# Autodesk Inventor assembly: CameraCaseMountV02
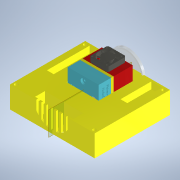
[picture p0: Inventor's stored thumbnail of the model, 180x180]
Saved by Autodesk Inventor 2022.2 (Build 262287000, 287)
## iProperties
Created: 2021-11-28
Part Number: CameraCaseMountV02
Document SubType Name: Assembly
Designer: robst
Author: robst
## Documents named in this file (4)
- C:\git\CAD-Development\robSteele\ShapeWays\GlobalMeteorNetwork\CameraCaseMountV02.iam
- C:\git\CAD-Development\robSteele\ShapeWays\GlobalMeteorNetwork\caseLowerPortionV02.ipt
- C:\git\CAD-Development\robSteele\ShapeWays\GlobalMeteorNetwork\IMX291 Camera Case Assembly.iam
- C:\git\CAD-Development\robSteele\ShapeWays\GlobalMeteorNetwork\50mmFilter.ipt
## Components (3 placed, 3 different names)
1. caseLowerPortionV02:1 — Mate:1, Mate:2, Mate:3, Insert:1
2. IMX291 Camera Case Assembly:1 [sub-assembly] — Mate:1, Mate:2, Mate:3
3. 50mmFilter:1 — Insert:1
## Relationships (4: Mate 3, Insert 1)
- Mate:1 (1 mm): caseLowerPortionV02:1 ↔ IMX291 Camera Case Assembly:1
- Mate:2 (1 mm): caseLowerPortionV02:1 ↔ IMX291 Camera Case Assembly:1
- Mate:3 (1 mm): caseLowerPortionV02:1 ↔ IMX291 Camera Case Assembly:1
- Insert:1: caseLowerPortionV02:1 ↔ 50mmFilter:1
